# Autodesk Inventor assembly: Vex Pulley 18 mm - 60T
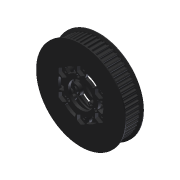
[picture p0: Inventor's stored thumbnail of the model, 180x180]
Saved by Autodesk Inventor 2013 (Build 170138000, 138)
## iProperties
Created: 2013-12-20
Part Number: Vex Pulley 18 mm - 60T
Document SubType Name: Assembly
Designer: Nemo
Author: Nemo
## Documents named in this file (3)
- H:\Nemo\Documents\Robotics\COTS Parts\Pulleys - Vex\Vex Pulley 18 mm - 60T.iam
- H:\Nemo\Documents\Robotics\COTS Parts\Pulleys - Vex\Components\Vex VersaPulley 60T half.ipt
- H:\Nemo\Documents\Robotics\COTS Parts\Pulleys - Vex\Components\Vex VersaPulley 60T center slice.ipt
## Components (3 placed, 2 different names)
1. Vex VersaPulley 60T half:1 — Mate:2, Flush:2, Mate:5
2. Vex VersaPulley 60T half:2 — Mate:3, Flush:3, Mate:6
3. Vex VersaPulley 60T center slice:1 — Mate:4, Mate:5, Mate:6, Flush:4
## Relationships (8: Mate 5, Flush 3)
- Mate:2: Vex VersaPulley 60T half:1
- Mate:3: Vex VersaPulley 60T half:2
- Flush:2: Vex VersaPulley 60T half:1
- Flush:3: Vex VersaPulley 60T half:2
- Mate:4: Vex VersaPulley 60T center slice:1
- Mate:5: Vex VersaPulley 60T half:1 ↔ Vex VersaPulley 60T center slice:1
- Mate:6: Vex VersaPulley 60T half:2 ↔ Vex VersaPulley 60T center slice:1
- Flush:4: Vex VersaPulley 60T center slice:1
